# Autodesk Inventor assembly: Assembly2
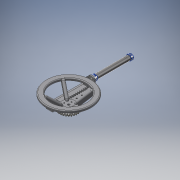
[picture p0: Inventor's stored thumbnail of the model, 180x180]
Saved by Autodesk Inventor 2017 (Build 210142000, 142)
## iProperties
Created: 2018-01-02
Part Number: Assembly2
Document SubType Name: Assembly
Designer: RLanting
Author: RLanting
## Documents named in this file (6)
- C:\Users\rmccomber\Documents\st motor\direct drive electronic valving 2\hydraulic steering\steering wheel\Assembly2.iam
- C:\Users\rmccomber\Documents\st motor\direct drive electronic valving 2\hydraulic steering\steering wheel\frame.ipt
- C:\Users\rmccomber\Documents\st motor\direct drive electronic valving 2\hydraulic steering\steering wheel\CJ2B16-100Z.iam
- C:\Users\rmccomber\Documents\st motor\direct drive electronic valving 2\hydraulic steering\steering wheel\Assembly2\Design Accelerator\Spur Gears2.iam
- C:\Users\rmccomber\Documents\st motor\direct drive electronic valving 2\hydraulic steering\steering wheel\rack.ipt
- C:\Users\rmccomber\Documents\st motor\direct drive electronic valving 2\hydraulic steering\steering wheel\steering wheel.ipt
## Components (5 placed, 5 different names)
1. frame:1 — Mate:1, Mate:2, Mate:3, Mate:4, Mate:5, Flush:1, Angle:1
2. CJ2B16-100Z:1 [sub-assembly] — Mate:1, Mate:2, Mate:6, Angle:1
3. Spur Gears:1 [sub-assembly] — Mate:3, Mate:4, Rotation/Translation:1, Mate:7, Mate:8, Mate:9
4. rack:1 — Mate:5, Flush:1, Mate:6, Rotation/Translation:1
5. steering wheel:1 — Mate:7, Mate:8, Mate:9
## Relationships (12: Mate 9, Flush 1, RelateRotateTranslate 1, Angle 1)
- Mate:1: frame:1 ↔ CJ2B16-100Z:1
- Mate:2: frame:1 ↔ CJ2B16-100Z:1
- Mate:3: frame:1 ↔ Spur Gears:1
- Mate:4: frame:1 ↔ Spur Gears:1
- Mate:5: frame:1 ↔ rack:1
- Flush:1 (-6 mm): frame:1 ↔ rack:1
- Mate:6: CJ2B16-100Z:1 ↔ rack:1
- Rotation/Translation:1 [RelateRotateTranslate] (197.82 mm): Spur Gears:1 ↔ rack:1
- Angle:1 (0 deg): frame:1 ↔ CJ2B16-100Z:1
- Mate:7: Spur Gears:1 ↔ steering wheel:1
- Mate:8: Spur Gears:1 ↔ steering wheel:1
- Mate:9: Spur Gears:1 ↔ steering wheel:1
